# Autodesk Inventor assembly: kinematicpairback
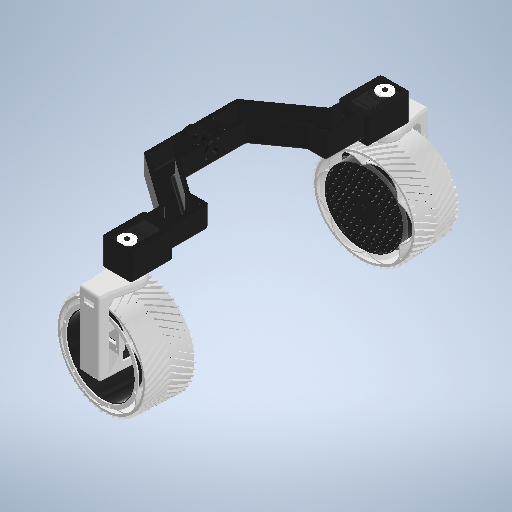
[picture p0: Inventor's stored thumbnail of the model, 512x512]
Saved by Autodesk Inventor 2025.3 (Build 293356000, 356)
## iProperties
Created: 2026-05-13
Part Number: kinematicpairback
Document SubType Name: Assembly
Designer: ksawe
Author: ksawe
## Documents named in this file (5)
- C:\Users\ksawe\OneDrive\Pulpit\Exomy v1\wersja3\kinematicpairback.iam
- C:\Users\ksawe\OneDrive\Pulpit\Exomy v1\wersja3\handler_back.ipt
- C:\Users\ksawe\OneDrive\Pulpit\Exomy v1\wersja3\basketback.ipt
- C:\Users\ksawe\OneDrive\Pulpit\Exomy v1\wersja3\serwo.iam
- C:\Users\ksawe\OneDrive\Pulpit\Exomy v1\wersja3\modul_napedowy.iam
## Components (7 placed, 4 different names)
1. handler_back:1 — Rigid:1, Rigid:2
2. basketback:1 — Rigid:1, Rigid:3
3. basketback:2 — Rigid:2, Rigid:4
4. serwo:1 [sub-assembly] — Rigid:4, Rigid:6
5. serwo:2 [sub-assembly] — Rigid:3, Rigid:5
6. modul_napedowy:1 [sub-assembly] — Rigid:5
7. modul_napedowy:2 [sub-assembly] — Rigid:6
## Relationships (6: WeldJoint 6)
- Rigid:1 [WeldJoint]: handler_back:1 ↔ basketback:1
- Rigid:2 [WeldJoint]: handler_back:1 ↔ basketback:2
- Rigid:3 [WeldJoint]: basketback:1 ↔ serwo:2
- Rigid:4 [WeldJoint]: basketback:2 ↔ serwo:1
- Rigid:5 [WeldJoint]: serwo:2 ↔ modul_napedowy:1
- Rigid:6 [WeldJoint]: serwo:1 ↔ modul_napedowy:2
